# Autodesk Inventor assembly: ASY GBK bottom 0021_CPY
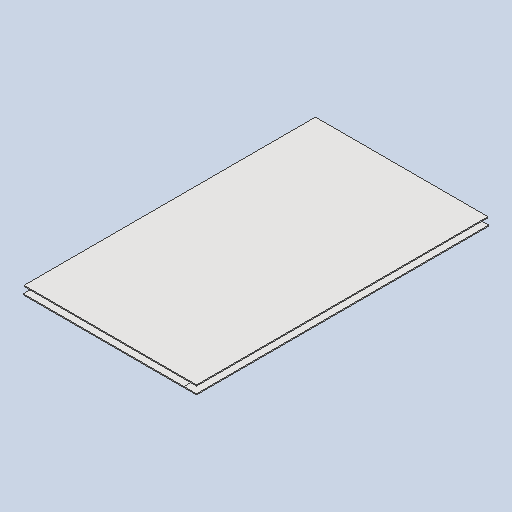
[picture p0: Inventor's stored thumbnail of the model, 512x512]
Saved by Autodesk Inventor 2026.2 (Build 302298000, 298)
## iProperties
Created: 2026-07-15
Part Number: ASY GBK bottom 0021_CPY
Document SubType Name: Assembly
Designer: user
Stock Number: 0060
Author: user
## Documents named in this file (4)
- C:\Users\admin\Documents\Inventor\GBK-Gubkinskiy\ASY GBK bottom 0021_CPY.iam
- C:\Users\admin\Documents\Inventor\GBK-Gubkinskiy\Пол\GBK bottom 0113_CPY.ipt
- C:\Users\admin\Documents\Inventor\GBK-Gubkinskiy\Пол\GBK bottom 0128_CPY.ipt
- C:\Users\admin\Documents\Inventor\GBK-Gubkinskiy\Пол\GBK bottom 0132_CPY.ipt
## Components (3 placed, 3 different names)
1. GBK bottom 0113_CPY:1 — Mate:3, Mate:2, Mate:1
2. GBK bottom 0128_CPY:1 — Mate:3, Rigid:1
3. GBK bottom 0132_CPY:1 — Mate:2, Mate:1, Rigid:1
## Relationships (4: Mate 3, WeldJoint 1)
- Mate:3 (-30 mm): GBK bottom 0113_CPY:1 ↔ GBK bottom 0128_CPY:1
- Mate:2 (-30 mm): GBK bottom 0113_CPY:1 ↔ GBK bottom 0132_CPY:1
- Mate:1: GBK bottom 0113_CPY:1 ↔ GBK bottom 0132_CPY:1
- Rigid:1 [WeldJoint]: GBK bottom 0128_CPY:1 ↔ GBK bottom 0132_CPY:1
